# Autodesk Inventor assembly: link assem
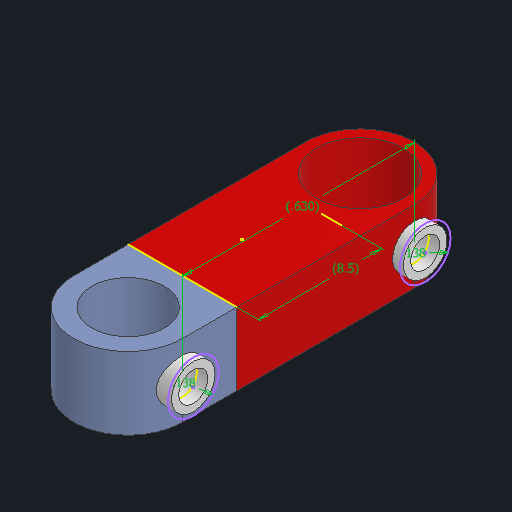
[picture p0: Inventor's stored thumbnail of the model, 512x512]
Saved by Autodesk Inventor 2025.1 (Build 291241000, 241)
## iProperties
Created: 2025-01-31
Part Number: link assem
Document SubType Name: Assembly
Designer: m_kni
Author: m_kni
## Documents named in this file (3)
- C:\Users\jerem\Documents\GitHub\Perovskite-Automated-Synthesis-System\CAD\Gripper\link assem.iam
- C:\Users\jerem\Documents\GitHub\Perovskite-Automated-Synthesis-System\CAD\Gripper\Link_InsideV3.ipt
- C:\Users\jerem\Documents\GitHub\Perovskite-Automated-Synthesis-System\CAD\Gripper\Link_OutsideV3.ipt
## Components (2 placed, 2 different names)
1. Link_InsideV3:1 — Mate:1, Flush:1, Flush:2
2. Link_OutsideV3:1 — Mate:1, Flush:1, Flush:2
## Relationships (3: Flush 2, Mate 1)
- Mate:1: Link_InsideV3:1 ↔ Link_OutsideV3:1
- Flush:1: Link_InsideV3:1 ↔ Link_OutsideV3:1
- Flush:2: Link_InsideV3:1 ↔ Link_OutsideV3:1
